# Autodesk Inventor assembly: Driver de Motor
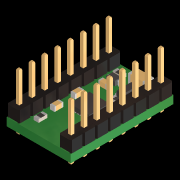
[picture p0: Inventor's stored thumbnail of the model, 180x180]
Saved by Autodesk Inventor 2022 (Build 260153000, 153)
## iProperties
Created: 2021-10-19
Part Number: Driver de Motor
Document SubType Name: Assembly
Designer: Julio R
Author: Julio R
## iProperties of the stored document 8x_Male_Pin_2.54_mm.iam
Created: 2020-05-13
Part Number: 8x_Male_Pin_2.54_mm
Description: STEP AP214
Document SubType Name: Assembly
Designer: Julio R
Title: 8x_Male_Pin_2.54_mm.STEP
Revision Number: ANY
Sending System: SolidWorks 2018
Preprocessor: SwSTEP 2.0
## iProperties of the stored document drv8833-dual-motor-driver-carrier-step.ipt
Created: 2018-11-02
Part Number: drv8833-dual-motor-driver-carrier-step
Material: Genérico
Description: STEP AP214
Document SubType Name: Modeling
Designer: Julio R
Density: 1 g/cm^3
Appearance: Valor por defecto
Title: drv8833-dual-motor-driver-carrier-step.step
Revision Number: ANY
Sending System: SolidWorks 2016
Preprocessor: SwSTEP 2.0
## iProperties of the stored document 1_Male_Pin_2.54_mm.ipt
Created: 2021-10-19
Part Number: 1_Male_Pin_2.54_mm
Material: Genérico
Document SubType Name: Modeling
Designer: Julio R
Density: 1 g/cm^3
Appearance: Valor por defecto
Author: Julio R
Revision Number: ANY
## Documents named in this file (6)
- **D:\Decimo Semestre\Diseño de Ingenieria\Diseño 3D\Driver de Motor.iam*LocalDocs*xAaaaq3aaAaaaaaaaAaaaae5vYe*8x_Male_Pin_2.54_mm.iam
- **D:\Decimo Semestre\Diseño de Ingenieria\Diseño 3D\Driver de Motor.iam*LocalDocs*xAaaaqucaAaaaaaaaAaaaq15bJc*1_Male_Pin_2.54_mm.ipt
- **D:\Decimo Semestre\Diseño de Ingenieria\Diseño 3D\Driver de Motor.iam*LocalDocs*xAaaaahcaAaaaaaaaAaaaqeslUh*drv8833-dual-motor-driver-carrier-step.ipt
- D:\Decimo Semestre\Diseño de Ingenieria\Diseño 3D\Driver de Motor.iam
- D:\Decimo Semestre\Diseño de Ingenieria\Diseño 3D\drv8833-dual-motor-driver-carrier-step.step
- D:\Decimo Semestre\Diseño de Ingenieria\Diseño 3D\headers-5.snapshot.1\8x_Male_Pin_2.54_mm.STEP
## Components (3 placed, 2 different names)
1. drv8833-dual-motor-driver-carrier-step:1 — Nivelación:1, Nivelación:2, Nivelación:3, Nivelación:4, Coincidencia:1, Coincidencia:2
2. 8x_Male_Pin_2.54_mm:1 [sub-assembly] — Nivelación:1, Nivelación:3, Coincidencia:1
3. 8x_Male_Pin_2.54_mm:2 [sub-assembly] — Nivelación:2, Nivelación:4, Coincidencia:2
## Relationships (6: Flush 4, Mate 2)
- Nivelación:1 [Flush]: drv8833-dual-motor-driver-carrier-step:1 ↔ 8x_Male_Pin_2.54_mm:1
- Nivelación:2 [Flush]: drv8833-dual-motor-driver-carrier-step:1 ↔ 8x_Male_Pin_2.54_mm:2
- Nivelación:3 [Flush]: drv8833-dual-motor-driver-carrier-step:1 ↔ 8x_Male_Pin_2.54_mm:1
- Nivelación:4 [Flush]: drv8833-dual-motor-driver-carrier-step:1 ↔ 8x_Male_Pin_2.54_mm:2
- Coincidencia:1 [Mate]: drv8833-dual-motor-driver-carrier-step:1 ↔ 8x_Male_Pin_2.54_mm:1
- Coincidencia:2 [Mate]: drv8833-dual-motor-driver-carrier-step:1 ↔ 8x_Male_Pin_2.54_mm:2
